# Autodesk Inventor assembly: Q.E
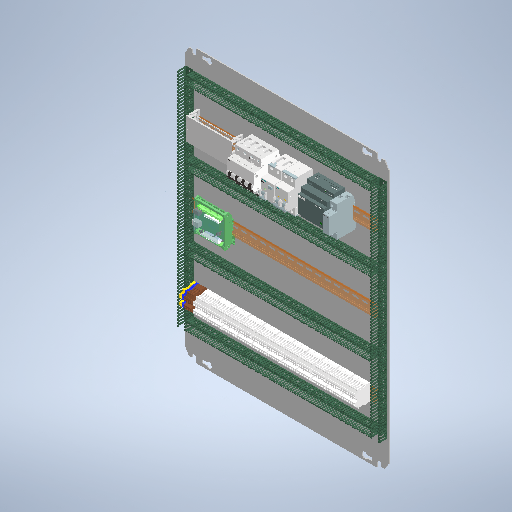
[picture p0: Inventor's stored thumbnail of the model, 512x512]
Saved by Autodesk Inventor 2025.2 (Build 292293000, 293)
## iProperties
Created: 2025-05-27
Part Number: Q.E
Document SubType Name: Assembly
Designer: Gustavo Sousa
Author: Gustavo Sousa
## Documents named in this file (16)
- C:\Users\lucas\OneDrive\Documentos\Documentos\Gustavo\Mozangao\Projeto Base (5140)\Q.E - Braço Robotico\Q.E_braco_robotico_9999_001.iam
- C:\Users\lucas\OneDrive\Documentos\Documentos\Gustavo\Mozangao\Projeto Base (5140)\Q.E - Braço Robotico\Q.E Rital\AIS2024\1376_000_1_\1376_000(1).iam
- C:\Users\lucas\OneDrive\Documentos\Documentos\Gustavo\Mozangao\Projeto Base (5140)\Q.E - Braço Robotico\CalhaDin\calhadin_001_0001.ipt
- C:\Users\lucas\OneDrive\Documentos\Documentos\Gustavo\Mozangao\Projeto Base (5140)\Q.E - Braço Robotico\CalhaPlastica\Calha_Plastica_40x40x1000_002_0001.ipt
- C:\Users\lucas\OneDrive\Documentos\Documentos\Gustavo\Mozangao\Projeto Base (5140)\Q.E - Braço Robotico\CalhaPlastica\Calha_Plastica_40x40x1000_001_0001.ipt
- C:\Users\lucas\OneDrive\Documentos\Documentos\Gustavo\Mozangao\Projeto Base (5140)\Q.E - Braço Robotico\Disjuntor Diferencial\disjuntor_diferencial_999_0001.iam
- C:\Users\lucas\OneDrive\Documentos\Documentos\Gustavo\Mozangao\Projeto Base (5140)\Q.E - Braço Robotico\Fonte de Alimentacao\f_alimentacao_230ac-5vdc_0001_001.iam
- C:\Users\lucas\OneDrive\Documentos\Documentos\Gustavo\Mozangao\Projeto Base (5140)\Q.E - Braço Robotico\Bornes Vikings\Bornes_Vikings_0001_001.ipt
- C:\Users\lucas\OneDrive\Documentos\Documentos\Gustavo\Mozangao\Projeto Base (5140)\Q.E - Braço Robotico\Bornes Vikings\Bornes_Vikings_0001_002.ipt
- C:\Users\lucas\OneDrive\Documentos\Documentos\Gustavo\Mozangao\Projeto Base (5140)\Q.E - Braço Robotico\Bornes Vikings\Bornes_Vikings_0001_003.ipt
- C:\Users\lucas\OneDrive\Documentos\Documentos\Gustavo\Mozangao\Projeto Base (5140)\Q.E - Braço Robotico\Disjuntor\disjuntor_bipolar_0001_001.ipt
- C:\Users\lucas\OneDrive\Documentos\Documentos\Gustavo\Mozangao\Projeto Base (5140)\Q.E - Braço Robotico\Bornes Vikings\Bornes_Vikings_0001_004.ipt
- C:\Users\lucas\OneDrive\Documentos\Documentos\Gustavo\Mozangao\Projeto Base (5140)\Q.E - Braço Robotico\Fusivel\Fusivel_0001_001.ipt
- C:\Users\lucas\OneDrive\Documentos\Documentos\Gustavo\Mozangao\Projeto Base (5140)\Q.E - Braço Robotico\Corte geral\Corte_geral_999_0001.iam
- C:\Users\lucas\OneDrive\Documentos\Documentos\Gustavo\Mozangao\Projeto Base (5140)\Q.E - Braço Robotico\Baramento escada\barramento_escada_0001_001.ipt
- C:\Users\lucas\OneDrive\Documentos\Documentos\Gustavo\Mozangao\Projeto Base (5140)\Q.E - Braço Robotico\Arduino\4556_ARDIUNO ADAPTER\4556_ARDIUNO ADAPTER\4556_ARDIUNO ADAPTER.ipt
## Components (88 placed, 15 different names)
1. 1376_000(1):1 [sub-assembly] — Alinhado:1, Alinhado:2, Alinhado:3, Coincidente:1, Coincidente:4, Coincidente:5, Coincidente:7, Coincidente:8, Coincidente:14, Coincidente:19, Coincidente:21, Alinhado:8, Coincidente:26, Coincidente:27, Coincidente:28, Coincidente:29, Coincidente:30, Coincidente:31, Coincidente:33
2. calhadin_001_0001 — Coincidente:1, Coincidente:4, Coincidente:6, Coincidente:7, Coincidente:9, Coincidente:10, Coincidente:23, Coincidente:34, Coincidente:35, Coincidente:36, Coincidente:37, Coincidente:46, Coincidente:47, Coincidente:74, Coincidente:75, Coincidente:76, Coincidente:77, Coincidente:78, Coincidente:79
3. calhadin_001_0001:2 — Coincidente:5, Coincidente:6, Coincidente:10, Alinhado:4, Alinhado:11, Coincidente:80, Coincidente:81
4. calhadin_001_0001:3 — Coincidente:8, Coincidente:9, Alinhado:4, Coincidente:40, Coincidente:41, Coincidente:42, Coincidente:43, Coincidente:44, Coincidente:45, Coincidente:48, Coincidente:49, Coincidente:58, Coincidente:59, Coincidente:64, Coincidente:65, Coincidente:67, Coincidente:68, Coincidente:69, Coincidente:70, Coincidente:71, Coincidente:72
5. Calha_Plastica_40x40x1000_002_0001 — Coincidente:14, Alinhado:6, Alinhado:8, Alinhado:9, Alinhado:10
6. Calha_Plastica_40x40x1000_002_0001:2 — Coincidente:19, Alinhado:6, Alinhado:10, Coincidente:32, Alinhado:12
7. Calha_Plastica_40x40x1000_002_0001:5 — Coincidente:21, Coincidente:23, Alinhado:9
8. Calha_Plastica_40x40x1000_001_0001:1 — Coincidente:26, Coincidente:27, Coincidente:28
9. Calha_Plastica_40x40x1000_001_0001:2 — Coincidente:29, Coincidente:30, Coincidente:31, Coincidente:32
10. Calha_Plastica_40x40x1000_002_0001:9 — Coincidente:33, Alinhado:11, Alinhado:12
11. disjuntor_diferencial_999_0001:1 [sub-assembly] — Coincidente:34, Coincidente:35
12. f_alimentacao_230ac-5vdc_0001_001:1 [sub-assembly] — Coincidente:36, Coincidente:37
13. Bornes_Vikings_0001_001:1 — Coincidente:40, Coincidente:41, Coincidente:50
14. Bornes_Vikings_0001_002:1 — Coincidente:44, Coincidente:45, Coincidente:50, Coincidente:57
15. disjuntor_bipolar_0001_001:1 — Coincidente:46, Coincidente:47
16. Fusivel_0001_001:1 — Coincidente:74, Coincidente:75
17. Corte_geral_999_0001:1 [sub-assembly] — Coincidente:76, Coincidente:77
18. barramento_escada_0001_001:1 — Coincidente:78, Coincidente:79
19. 4556_ARDIUNO ADAPTER:1 — Coincidente:80, Coincidente:81
20. Bornes_Vikings_0001_004:1 — Coincidente:48, Coincidente:49, Coincidente:60
21. Bornes_Vikings_0001_004:2 — Coincidente:58, Coincidente:59, Coincidente:60, Coincidente:66
22. Bornes_Vikings_0001_004:4 — Coincidente:61, Coincidente:62, Coincidente:67, Coincidente:68
23. Bornes_Vikings_0001_004:3 — Coincidente:61, Coincidente:64, Coincidente:65, Coincidente:66
24. Bornes_Vikings_0001_004:6 — Coincidente:63, Coincidente:71, Coincidente:72
25. Bornes_Vikings_0001_004:5 — Coincidente:62, Coincidente:63, Coincidente:69, Coincidente:70
26. Bornes_Vikings_0001_004:7
27. Bornes_Vikings_0001_004:8
28. Bornes_Vikings_0001_004:9
29. Bornes_Vikings_0001_004:10
30. Bornes_Vikings_0001_004:11
31. Bornes_Vikings_0001_004:12
32. Bornes_Vikings_0001_004:13
33. Bornes_Vikings_0001_004:14
34. Bornes_Vikings_0001_004:15
35. Bornes_Vikings_0001_004:16
36. Bornes_Vikings_0001_004:17
37. Bornes_Vikings_0001_004:18
38. Bornes_Vikings_0001_004:19
39. Bornes_Vikings_0001_004:20
40. Bornes_Vikings_0001_004:21
41. Bornes_Vikings_0001_004:22
42. Bornes_Vikings_0001_004:23
43. Bornes_Vikings_0001_004:24
44. Bornes_Vikings_0001_004:25
45. Bornes_Vikings_0001_004:26
46. Bornes_Vikings_0001_004:27
47. Bornes_Vikings_0001_004:28
48. Bornes_Vikings_0001_004:29
49. Bornes_Vikings_0001_004:30
50. Bornes_Vikings_0001_004:31
51. Bornes_Vikings_0001_004:32
52. Bornes_Vikings_0001_004:33
53. Bornes_Vikings_0001_004:34
54. Bornes_Vikings_0001_004:35
55. Bornes_Vikings_0001_004:36
56. Bornes_Vikings_0001_004:37
57. Bornes_Vikings_0001_004:38
58. Bornes_Vikings_0001_004:39
59. Bornes_Vikings_0001_004:40
60. Bornes_Vikings_0001_004:41
61. Bornes_Vikings_0001_004:42
62. Bornes_Vikings_0001_004:43
63. Bornes_Vikings_0001_004:44
64. Bornes_Vikings_0001_004:45
65. Bornes_Vikings_0001_004:46
66. Bornes_Vikings_0001_004:47
67. Bornes_Vikings_0001_004:48
68. Bornes_Vikings_0001_004:49
69. Bornes_Vikings_0001_004:50
70. Bornes_Vikings_0001_004:51
71. Bornes_Vikings_0001_004:52
72. Bornes_Vikings_0001_004:53
73. Bornes_Vikings_0001_004:54
74. Bornes_Vikings_0001_004:55
75. Bornes_Vikings_0001_004:56
76. Bornes_Vikings_0001_004:57
77. Bornes_Vikings_0001_004:58
78. Bornes_Vikings_0001_004:59
79. Bornes_Vikings_0001_004:60
80. Bornes_Vikings_0001_004:61
81. Bornes_Vikings_0001_004:62
82. Bornes_Vikings_0001_004:63
83. Bornes_Vikings_0001_004:64
84. Bornes_Vikings_0001_004:65
85. Bornes_Vikings_0001_004:66
86. Bornes_Vikings_0001_003:1 — Coincidente:42, Coincidente:43, Coincidente:57
87. Bornes_Vikings_0001_003:2
88. Bornes_Vikings_0001_003:3
## Component patterns: (11 elements, first: Bornes_Vikings_0001_004:1 + Bornes_Vikings_0001_004:2 + Bornes_Vikings_0001_004:4 + Bornes_Vikings_0001_004:3 + Bornes_Vikings_0001_004:6 + Bornes_Vikings_0001_004:5), (3 elements, first: Bornes_Vikings_0001_003:1)
## Relationships (69: Mate 59, Flush 10)
- Alinhado:1 [Flush]: 1376_000(1):1
- Alinhado:2 [Flush]: 1376_000(1):1
- Alinhado:3 [Flush]: 1376_000(1):1
- Coincidente:1 [Mate]: 1376_000(1):1 ↔ calhadin_001_0001
- Coincidente:4 [Mate] (558 mm): 1376_000(1):1 ↔ calhadin_001_0001
- Coincidente:5 [Mate]: 1376_000(1):1 ↔ calhadin_001_0001:2
- Coincidente:6 [Mate]: calhadin_001_0001 ↔ calhadin_001_0001:2
- Coincidente:7 [Mate]: 1376_000(1):1 ↔ calhadin_001_0001
- Coincidente:8 [Mate]: 1376_000(1):1 ↔ calhadin_001_0001:3
- Coincidente:9 [Mate]: calhadin_001_0001 ↔ calhadin_001_0001:3
- Coincidente:10 [Mate] (199 mm): calhadin_001_0001 ↔ calhadin_001_0001:2
- Alinhado:4 [Flush] (199 mm): calhadin_001_0001:2 ↔ calhadin_001_0001:3
- Coincidente:14 [Mate]: 1376_000(1):1 ↔ Calha_Plastica_40x40x1000_002_0001
- Coincidente:19 [Mate]: 1376_000(1):1 ↔ Calha_Plastica_40x40x1000_002_0001:2
- Alinhado:6 [Flush] (574.5 mm): Calha_Plastica_40x40x1000_002_0001 ↔ Calha_Plastica_40x40x1000_002_0001:2
- Coincidente:21 [Mate]: 1376_000(1):1 ↔ Calha_Plastica_40x40x1000_002_0001:5
- Coincidente:23 [Mate] (99.5 mm): calhadin_001_0001 ↔ Calha_Plastica_40x40x1000_002_0001:5
- Alinhado:8 [Flush] (-657.5 mm): 1376_000(1):1 ↔ Calha_Plastica_40x40x1000_002_0001
- Coincidente:26 [Mate]: 1376_000(1):1 ↔ Calha_Plastica_40x40x1000_001_0001:1
- Coincidente:27 [Mate] (370 mm): 1376_000(1):1 ↔ Calha_Plastica_40x40x1000_001_0001:1
- Coincidente:28 [Mate] (2.2 mm): 1376_000(1):1 ↔ Calha_Plastica_40x40x1000_001_0001:1
- Coincidente:29 [Mate]: 1376_000(1):1 ↔ Calha_Plastica_40x40x1000_001_0001:2
- Coincidente:30 [Mate] (370 mm): 1376_000(1):1 ↔ Calha_Plastica_40x40x1000_001_0001:2
- Coincidente:31 [Mate] (2.2 mm): 1376_000(1):1 ↔ Calha_Plastica_40x40x1000_001_0001:2
- Alinhado:9 [Flush]: Calha_Plastica_40x40x1000_002_0001 ↔ Calha_Plastica_40x40x1000_002_0001:5
- Alinhado:10 [Flush]: Calha_Plastica_40x40x1000_002_0001 ↔ Calha_Plastica_40x40x1000_002_0001:2
- Coincidente:32 [Mate] (1.7 mm): Calha_Plastica_40x40x1000_002_0001:2 ↔ Calha_Plastica_40x40x1000_001_0001:2
- Coincidente:33 [Mate]: 1376_000(1):1 ↔ Calha_Plastica_40x40x1000_002_0001:9
- Alinhado:11 [Flush] (99.5 mm): calhadin_001_0001:2 ↔ Calha_Plastica_40x40x1000_002_0001:9
- Alinhado:12 [Flush]: Calha_Plastica_40x40x1000_002_0001:2 ↔ Calha_Plastica_40x40x1000_002_0001:9
- Coincidente:34 [Mate]: calhadin_001_0001 ↔ disjuntor_diferencial_999_0001:1
- Coincidente:35 [Mate]: calhadin_001_0001 ↔ disjuntor_diferencial_999_0001:1
- Coincidente:36 [Mate]: calhadin_001_0001 ↔ f_alimentacao_230ac-5vdc_0001_001:1
- Coincidente:37 [Mate]: calhadin_001_0001 ↔ f_alimentacao_230ac-5vdc_0001_001:1
- Coincidente:40 [Mate]: calhadin_001_0001:3 ↔ Bornes_Vikings_0001_001:1
- Coincidente:41 [Mate]: calhadin_001_0001:3 ↔ Bornes_Vikings_0001_001:1
- Coincidente:42 [Mate]: calhadin_001_0001:3 ↔ Bornes_Vikings_0001_003:1
- Coincidente:43 [Mate]: calhadin_001_0001:3 ↔ Bornes_Vikings_0001_003:1
- Coincidente:44 [Mate]: calhadin_001_0001:3 ↔ Bornes_Vikings_0001_002:1
- Coincidente:45 [Mate]: calhadin_001_0001:3 ↔ Bornes_Vikings_0001_002:1
- Coincidente:46 [Mate]: calhadin_001_0001 ↔ disjuntor_bipolar_0001_001:1
- Coincidente:47 [Mate]: calhadin_001_0001 ↔ disjuntor_bipolar_0001_001:1
- Coincidente:48 [Mate]: calhadin_001_0001:3 ↔ Bornes_Vikings_0001_004:1
- Coincidente:49 [Mate]: calhadin_001_0001:3 ↔ Bornes_Vikings_0001_004:1
- Coincidente:50 [Mate]: Bornes_Vikings_0001_001:1 ↔ Bornes_Vikings_0001_002:1
- Coincidente:57 [Mate]: Bornes_Vikings_0001_002:1 ↔ Bornes_Vikings_0001_003:1
- Coincidente:58 [Mate]: calhadin_001_0001:3 ↔ Bornes_Vikings_0001_004:2
- Coincidente:59 [Mate]: calhadin_001_0001:3 ↔ Bornes_Vikings_0001_004:2
- Coincidente:60 [Mate]: Bornes_Vikings_0001_004:1 ↔ Bornes_Vikings_0001_004:2
- Coincidente:61 [Mate]: Bornes_Vikings_0001_004:4 ↔ Bornes_Vikings_0001_004:3
- Coincidente:62 [Mate]: Bornes_Vikings_0001_004:4 ↔ Bornes_Vikings_0001_004:5
- Coincidente:63 [Mate]: Bornes_Vikings_0001_004:6 ↔ Bornes_Vikings_0001_004:5
- Coincidente:64 [Mate]: calhadin_001_0001:3 ↔ Bornes_Vikings_0001_004:3
- Coincidente:65 [Mate]: calhadin_001_0001:3 ↔ Bornes_Vikings_0001_004:3
- Coincidente:66 [Mate]: Bornes_Vikings_0001_004:2 ↔ Bornes_Vikings_0001_004:3
- Coincidente:67 [Mate]: calhadin_001_0001:3 ↔ Bornes_Vikings_0001_004:4
- Coincidente:68 [Mate]: calhadin_001_0001:3 ↔ Bornes_Vikings_0001_004:4
- Coincidente:69 [Mate]: calhadin_001_0001:3 ↔ Bornes_Vikings_0001_004:5
- Coincidente:70 [Mate]: calhadin_001_0001:3 ↔ Bornes_Vikings_0001_004:5
- Coincidente:71 [Mate]: calhadin_001_0001:3 ↔ Bornes_Vikings_0001_004:6
- Coincidente:72 [Mate]: calhadin_001_0001:3 ↔ Bornes_Vikings_0001_004:6
- Coincidente:74 [Mate]: calhadin_001_0001 ↔ Fusivel_0001_001:1
- Coincidente:75 [Mate]: calhadin_001_0001 ↔ Fusivel_0001_001:1
- Coincidente:76 [Mate]: calhadin_001_0001 ↔ Corte_geral_999_0001:1
- Coincidente:77 [Mate]: calhadin_001_0001 ↔ Corte_geral_999_0001:1
- Coincidente:78 [Mate]: calhadin_001_0001 ↔ barramento_escada_0001_001:1
- Coincidente:79 [Mate]: calhadin_001_0001 ↔ barramento_escada_0001_001:1
- Coincidente:80 [Mate]: calhadin_001_0001:2 ↔ 4556_ARDIUNO ADAPTER:1
- Coincidente:81 [Mate]: calhadin_001_0001:2 ↔ 4556_ARDIUNO ADAPTER:1
